# Autodesk Inventor assembly: cabeça_superior3
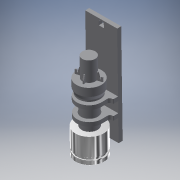
[picture p0: Inventor's stored thumbnail of the model, 180x180]
Saved by Autodesk Inventor 2018 (Build 220112000, 112)
## iProperties
Created: 2018-05-10
Part Number: cabeça_superior3
Material: Genérico
Document SubType Name: Assembly
Designer: Georgines
Mass: 943.179 g
Surface Area: 3340.88 cm^2
Volume: 704.097 cm^3
Density: 1.33956 g/cm^3
Author: Georgines
## Documents named in this file (6)
- C:\Users\Usuario\Desktop\Estação BGA\Peças 3D\cabeça_superior3.iam
- C:\Users\Usuario\Desktop\Estação BGA\Peças 3D\bocal_de_aquecimento.ipt
- C:\Users\Usuario\Desktop\Estação BGA\Peças 3D\soprador_original.ipt
- C:\Users\Usuario\Desktop\Estação BGA\Peças 3D\base_fixaxao_cabeca_supeior.ipt
- C:\Users\Usuario\Desktop\Estação BGA\Peças 3D\carcaca_bocal_superior.ipt
- C:\Users\Usuario\Desktop\Estação BGA\Peças 3D\SuporteAquecedor.ipt
## Components (6 placed, 5 different names)
1. bocal_de_aquecimento:1 — Coincidência:16, Alinhamento:14, Coincidência:22
2. soprador_original:1 — Coincidência:15, Coincidência:16, Alinhamento:14, Coincidência:17
3. base_fixaxao_cabeca_supeior:1 — Coincidência:12, Alinhamento:10, Coincidência:13, Alinhamento:11, Alinhamento:12, Coincidência:18, Alinhamento:15, Coincidência:22
4. SuporteAquecedor:1 — Coincidência:12, Alinhamento:10, Alinhamento:12, Coincidência:14, Coincidência:15, Coincidência:17
5. SuporteAquecedor:2 — Coincidência:13, Alinhamento:11, Coincidência:14
6. carcaca_bocal_superior:1 — Coincidência:18, Alinhamento:15
## Relationships (13: Mate 8, Flush 5)
- Coincidência:12 [Mate]: base_fixaxao_cabeca_supeior:1 ↔ SuporteAquecedor:1
- Alinhamento:10 [Flush]: base_fixaxao_cabeca_supeior:1 ↔ SuporteAquecedor:1
- Coincidência:13 [Mate]: base_fixaxao_cabeca_supeior:1 ↔ SuporteAquecedor:2
- Alinhamento:11 [Flush]: base_fixaxao_cabeca_supeior:1 ↔ SuporteAquecedor:2
- Alinhamento:12 [Flush] (142.072 mm): base_fixaxao_cabeca_supeior:1 ↔ SuporteAquecedor:1
- Coincidência:14 [Mate] (25.75 mm): SuporteAquecedor:1 ↔ SuporteAquecedor:2
- Coincidência:15 [Mate]: soprador_original:1 ↔ SuporteAquecedor:1
- Coincidência:16 [Mate]: bocal_de_aquecimento:1 ↔ soprador_original:1
- Alinhamento:14 [Flush] (2.5 mm): bocal_de_aquecimento:1 ↔ soprador_original:1
- Coincidência:17 [Mate] (5 mm): soprador_original:1 ↔ SuporteAquecedor:1
- Coincidência:18 [Mate]: base_fixaxao_cabeca_supeior:1 ↔ carcaca_bocal_superior:1
- Alinhamento:15 [Flush]: base_fixaxao_cabeca_supeior:1 ↔ carcaca_bocal_superior:1
- Coincidência:22 [Mate]: bocal_de_aquecimento:1 ↔ base_fixaxao_cabeca_supeior:1
